# Autodesk Inventor assembly: Assembly1
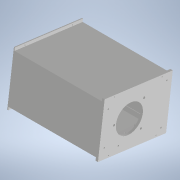
[picture p0: Inventor's stored thumbnail of the model, 180x180]
Saved by Autodesk Inventor 2020.3 (Build 243373000, 373)
## iProperties
Created: 2020-08-18
Part Number: Assembly1
Document SubType Name: Assembly
Designer: joesp
Author: joesp
## Documents named in this file (6)
- C:\Users\joesp\Desktop\fullmotion racing sim\Steering Wheel\3d models\Assembly1.iam
- C:\Users\joesp\Desktop\fullmotion racing sim\Steering Wheel\3d models\shell.ipt
- C:\Users\joesp\Desktop\fullmotion racing sim\Steering Wheel\3d models\front plate.ipt
- C:\Users\joesp\Desktop\fullmotion racing sim\Steering Wheel\3d models\IRSensorMount.ipt
- C:\Users\joesp\Desktop\fullmotion racing sim\Steering Wheel\3d models\IRSensorMountOtherSide.ipt
- C:\Users\joesp\Desktop\fullmotion racing sim\Steering Wheel\3d models\back plate.ipt
## Components (5 placed, 5 different names)
1. shell:1 — Mate:1, Mate:2, Mate:3, Mate:8, Flush:1
2. front plate:1 — Mate:1, Mate:2, Mate:3, Mate:4, Mate:5, Mate:6, Mate:7, Mate:9
3. IRSensorMount:1 — Mate:4, Mate:5
4. IRSensorMountOtherSide:1 — Mate:6, Mate:7
5. back plate:1 — Mate:8, Flush:1, Mate:9
## Relationships (10: Mate 9, Flush 1)
- Mate:1: shell:1 ↔ front plate:1
- Mate:2: shell:1 ↔ front plate:1
- Mate:3: shell:1 ↔ front plate:1
- Mate:4: front plate:1 ↔ IRSensorMount:1
- Mate:5: front plate:1 ↔ IRSensorMount:1
- Mate:6: front plate:1 ↔ IRSensorMountOtherSide:1
- Mate:7: front plate:1 ↔ IRSensorMountOtherSide:1
- Mate:8: shell:1 ↔ back plate:1
- Flush:1: shell:1 ↔ back plate:1
- Mate:9: front plate:1 ↔ back plate:1
